# Autodesk Inventor assembly: Assembly1
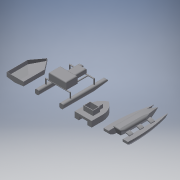
[picture p0: Inventor's stored thumbnail of the model, 180x180]
Saved by Autodesk Inventor 2016 (Build 200138000, 138)
## iProperties
Created: 2019-01-14
Part Number: Assembly1
Document SubType Name: Assembly
Designer: LinJie
Author: LinJie
## Documents named in this file (5)
- C:\Users\LinJie\Documents\Inventor\EA Water project\Assembly1.iam
- C:\Users\LinJie\Documents\Inventor\EA Water project\Generalcraftshape1.ipt
- C:\Users\LinJie\Documents\Inventor\EA Water project\GeneralCraftShape2.ipt
- C:\Users\LinJie\Documents\Inventor\EA Water project\GeneralCraftShape3.ipt
- C:\Users\LinJie\Documents\Inventor\EA Water project\GeneralCraftShape4.ipt
## Components (4 placed, 4 different names)
1. Generalcraftshape1:1 — Mate:1, Flush:1, Flush:2
2. GeneralCraftShape2:1 — Mate:1, Flush:1, Flush:2, Mate:2, Flush:3, Flush:4
3. GeneralCraftShape3:1 — Mate:2, Flush:3, Flush:4, Flush:5, Flush:6, Mate:3
4. GeneralCraftShape4:1 — Flush:5, Flush:6, Mate:3
## Relationships (9: Flush 6, Mate 3)
- Mate:1 (200 mm): Generalcraftshape1:1 ↔ GeneralCraftShape2:1
- Flush:1: Generalcraftshape1:1 ↔ GeneralCraftShape2:1
- Flush:2: Generalcraftshape1:1 ↔ GeneralCraftShape2:1
- Mate:2 (200 mm): GeneralCraftShape2:1 ↔ GeneralCraftShape3:1
- Flush:3: GeneralCraftShape2:1 ↔ GeneralCraftShape3:1
- Flush:4: GeneralCraftShape2:1 ↔ GeneralCraftShape3:1
- Flush:5: GeneralCraftShape3:1 ↔ GeneralCraftShape4:1
- Flush:6: GeneralCraftShape3:1 ↔ GeneralCraftShape4:1
- Mate:3 (300 mm): GeneralCraftShape3:1 ↔ GeneralCraftShape4:1
